# Autodesk Inventor assembly: VersaPlanetary_2stg_dual-775
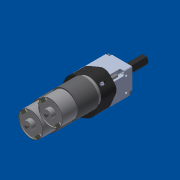
[picture p0: Inventor's stored thumbnail of the model, 180x180]
Saved by Autodesk Inventor 2016 (Build 200138000, 138)
## iProperties
Created: 2016-01-31
Part Number: VersaPlanetary_2stg_dual-775
Document SubType Name: Assembly
Designer: Beezy
Author: Beezy
## Documents named in this file (3)
- C:\Users\FIRSTUser\Documents\GrabCAD\2016 Robot\Imported Components\Gearboxes\VersaPlanetary_2stg_dual-775.iam
- C:\Users\FIRSTUser\Documents\GrabCAD\2016 Robot\Imported Components\Gearboxes\VersaPlanetary_2stg_775.ipt
- C:\Users\FIRSTUser\Documents\GrabCAD\2016 Robot\Imported Components\Gearboxes\VersaPlanetary_Dual-775.iam
## Components (2 placed, 2 different names)
1. VersaPlanetary_2stg_775:1 — Mate:1, Mate:2, Mate:3
2. VersaPlanetary_Dual-775:1 [sub-assembly] — Mate:1, Mate:2, Mate:3
## Relationships (3: Mate 3)
- Mate:1: VersaPlanetary_2stg_775:1 ↔ VersaPlanetary_Dual-775:1
- Mate:2: VersaPlanetary_2stg_775:1 ↔ VersaPlanetary_Dual-775:1
- Mate:3 (-16.8148 mm): VersaPlanetary_2stg_775:1 ↔ VersaPlanetary_Dual-775:1
